# Autodesk Inventor assembly: False_Bottom_Geared_2
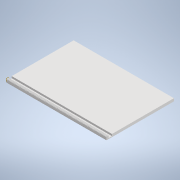
[picture p0: Inventor's stored thumbnail of the model, 180x180]
Saved by Autodesk Inventor 2020 (Build 240168000, 168)
## iProperties
Created: 2022-01-22
Part Number: False_Bottom_Geared_2
Document SubType Name: Assembly
Designer: danie
Author: danie
## Documents named in this file (3)
- C:\Users\danie\Documents\Capstone\Solidworks\False_Bottom_Geared_2.iam
- C:\Users\danie\Documents\Capstone\Solidworks\False_Bottom_4.ipt
- C:\Users\danie\Documents\Capstone\Solidworks\2662N54_20 Degree Pressure Angle Gear Rack_2.ipt
## Components (2 placed, 2 different names)
1. False_Bottom_4:1 — Rigid:1
2. 2662N54_20 Degree Pressure Angle Gear Rack_2:1 — Rigid:1
## Relationships (1: WeldJoint 1)
- Rigid:1 [WeldJoint]: False_Bottom_4:1 ↔ 2662N54_20 Degree Pressure Angle Gear Rack_2:1
